# Autodesk Inventor assembly: Asem
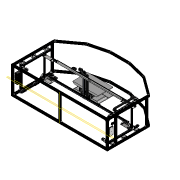
[picture p0: Inventor's stored thumbnail of the model, 180x180]
Saved by Autodesk Inventor 2020 (Build 240168000, 168)
## iProperties
Created: 2021-02-24
Part Number: Asem
Document SubType Name: Assembly
Designer: magnarecta
Author: magnarecta
## Documents named in this file (7)
- D:\Documents\GitHub\Eto_Project\Hardware\Asem\Asem.iam
- D:\Documents\GitHub\Eto_Project\Hardware\Asem\CCM_Unit.iam
- D:\Documents\GitHub\Eto_Project\Hardware\Asem\Display_Unit.iam
- D:\Documents\GitHub\Eto_Project\Hardware\Parts\Grabcad\nema-23-stepper-motors-driver-1.snapshot.7\DM542T Digital Stepper Drive.ipt
- D:\Documents\GitHub\Eto_Project\Hardware\Parts\Grabcad\mean-well-lrs-350-24-1.snapshot.3\meanwell_lrs-350-24_UPDATED.ipt
- D:\Documents\GitHub\Eto_Project\Hardware\Parts\Grabcad\ac-power-switch-assembly-1.snapshot.2\AC Power Switch Assy.iam
- D:\Documents\GitHub\Eto_Project\Hardware\Parts\MISUMI_FRAMES\model_ver4\1208.iam
## Components (13 placed, 6 different names)
1. CCM_Unit:1 [sub-assembly] — 挿入:1, 挿入:2, フラッシュ:5, メイト:4, フラッシュ:6
2. Display_Unit:1 [sub-assembly] — 挿入:1, 挿入:2
3. meanwell_lrs-350-24_UPDATED:1
4. AC Power Switch Assy:1 [sub-assembly] — フラッシュ:3
5. AC Power Switch Assy:2 [sub-assembly] — フラッシュ:3
6. 1208:1 [sub-assembly] — メイト:1, メイト:2, メイト:3, フラッシュ:5, メイト:4, フラッシュ:6
7. DM542T Digital Stepper Drive:1
8. DM542T Digital Stepper Drive:2
9. DM542T Digital Stepper Drive:3
10. DM542T Digital Stepper Drive:4
11. DM542T Digital Stepper Drive:5
12. DM542T Digital Stepper Drive:6
13. DM542T Digital Stepper Drive:7
## Component patterns: (7 elements, first: DM542T Digital Stepper Drive:1)
## Relationships (9: Mate 4, Flush 3, Insert 2)
- 挿入:1 [Insert]: CCM_Unit:1 ↔ Display_Unit:1
- フラッシュ:3 [Flush]: AC Power Switch Assy:1 ↔ AC Power Switch Assy:2
- 挿入:2 [Insert]: CCM_Unit:1 ↔ Display_Unit:1
- メイト:1 [Mate]: 1208:1
- メイト:2 [Mate] (-1400 mm): 1208:1
- メイト:3 [Mate] (355 mm): 1208:1
- フラッシュ:5 [Flush]: CCM_Unit:1 ↔ 1208:1
- メイト:4 [Mate]: CCM_Unit:1 ↔ 1208:1
- フラッシュ:6 [Flush]: CCM_Unit:1 ↔ 1208:1
